# Autodesk Inventor assembly: Zespół tłoka
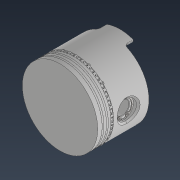
[picture p0: Inventor's stored thumbnail of the model, 180x180]
Saved by Autodesk Inventor 2022 (Build 260153000, 153)
## iProperties
Created: 2023-05-22
Part Number: Zespół tłoka
Document SubType Name: Assembly
Designer: wikto
Author: wikto
## Documents named in this file (7)
- C:\Users\wikto\Desktop\Inventor - szkoła\Boxer Garbus\Zespół tłoka.iam
- C:\Users\wikto\Desktop\Inventor - szkoła\Boxer Garbus\Tłok.ipt
- C:\Users\wikto\Desktop\Inventor - szkoła\Boxer Garbus\Pierścień zgarniający, zgarniająco-kompensacyjny.ipt
- C:\Users\wikto\Desktop\Inventor - szkoła\Boxer Garbus\Pierścień zgarniający.ipt
- C:\Users\wikto\Desktop\Inventor - szkoła\Boxer Garbus\Pierścień uszczelniający tłoka.ipt
- C:\Users\wikto\Desktop\Inventor - szkoła\Boxer Garbus\Sworzeń tłoka.ipt
- C:\Users\wikto\OneDrive\Documents\Inventor\Content Center Files\R2022\en-US\BS 3673(7)\BS 3673_ Part 4 - B022 M.ipt
## Components (7 placed, 6 different names)
1. Tłok:1 — Mate:1, Mate:2, Mate:3, Mate:4, Mate:5, Mate:6, Insert:1, Insert:2, Insert:3
2. Pierścień zgarniający, zgarniająco-kompensacyjny:1 — Mate:3, Mate:4
3. Pierścień zgarniający:1 — Mate:1, Mate:2
4. Pierścień uszczelniający tłoka:1 — Mate:5, Mate:6
5. Sworzeń tłoka:1 — Insert:1
6. BS 3673 : Part 4 - Metric B022 M:1 — Insert:2
7. BS 3673 : Part 4 - Metric B022 M:2 — Insert:3
## Relationships (9: Mate 6, Insert 3)
- Mate:1: Tłok:1 ↔ Pierścień zgarniający:1
- Mate:2: Tłok:1 ↔ Pierścień zgarniający:1
- Mate:3: Tłok:1 ↔ Pierścień zgarniający, zgarniająco-kompensacyjny:1
- Mate:4: Tłok:1 ↔ Pierścień zgarniający, zgarniająco-kompensacyjny:1
- Mate:5: Tłok:1 ↔ Pierścień uszczelniający tłoka:1
- Mate:6: Tłok:1 ↔ Pierścień uszczelniający tłoka:1
- Insert:1: Tłok:1 ↔ Sworzeń tłoka:1
- Insert:2: Tłok:1 ↔ BS 3673 : Part 4 - Metric B022 M:1
- Insert:3: Tłok:1 ↔ BS 3673 : Part 4 - Metric B022 M:2
